# Autodesk Inventor assembly: Sestava1
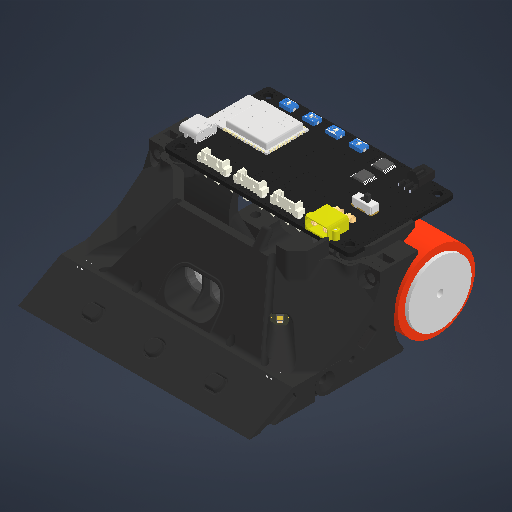
[picture p0: Inventor's stored thumbnail of the model, 512x512]
Saved by Autodesk Inventor 2025 (Build 290162000, 162)
## iProperties
Created: 2024-10-19
Part Number: Sestava1
Document SubType Name: Assembly
Designer: Simak
Author: Simak
## Documents named in this file (12)
- C:\_desktop\GitHub\Sumec-MiniSumo\-3D-\main_sumec_assembly.iam
- C:\_desktop\GitHub\Sumec-MiniSumo\-3D-\3D_printed\body-main.ipt
- C:\_desktop\GitHub\Sumec-MiniSumo\-3D-\3D_printed\body-front.ipt
- C:\_desktop\GitHub\Sumec-MiniSumo\-3D-\electronics\pololu-digital-distance-sensor-irs17a.ipt
- C:\_desktop\GitHub\Sumec-MiniSumo\-3D-\electronics\AssemBeneWake TF-LUNA.ipt
- C:\_desktop\GitHub\Sumec-MiniSumo\-3D-\electronics\PCBs\QRE MiniBoards\QRE MiniBoards\QRE_MiniBoards_Board.iam
- C:\_desktop\GitHub\Sumec-MiniSumo\-3D-\3D_printed\body-motor_comparment.ipt
- C:\_desktop\GitHub\Sumec-MiniSumo\-3D-\electronics\pololu_12v_650rpm-cb-enc-side-con.ipt
- C:\_desktop\GitHub\Sumec-MiniSumo\-3D-\machined\JSUMO_Wheel_33x25mm.ipt
- C:\_desktop\GitHub\Sumec-MiniSumo\-3D-\3D_printed\motor_C_clamp.ipt
- C:\_desktop\GitHub\Sumec-MiniSumo\-3D-\electronics\PCBs\main board\SUMEC_MK_IV.iam
- C:\_desktop\GitHub\Sumec-MiniSumo\-3D-\electronics\3s_lipo_small.ipt
## Components (12 placed, 11 different names)
1. body-main:1 — OPEN, Stejný směr:1, Vložit:1, Vložit:3, Proti sobě:6, Stejný směr:3, Proti sobě:7, Stejný směr:5, Vložit:6, Stejný směr:7, Vložit:7
2. body-front:1 — OPEN, Stejný směr:1, Vložit:1, Stejný směr:2, Proti sobě:2, Proti sobě:3, Proti sobě:4, Úhel:1, Tečnost:1, Vložit:2, Proti sobě:5
3. pololu-digital-distance-sensor-irs17a:1 — Stejný směr:2, Proti sobě:2, Proti sobě:3
4. AssemBeneWake TF-LUNA:1 — Proti sobě:4, Úhel:1, Tečnost:1
5. QRE_MiniBoards_Board:1 [sub-assembly] — Vložit:2, Proti sobě:5
6. pololu-digital-distance-sensor-irs17a:2 — Vložit:3, Proti sobě:6
7. body-motor_comparment:1 — Stejný směr:3, Proti sobě:7, Proti sobě:8, Proti sobě:9, Proti sobě:10, Proti sobě:11, Vložit:5, Stejný směr:6, Vložit:7
8. pololu_12v_650rpm-cb-enc-side-con:1 — Proti sobě:8, Proti sobě:9, Proti sobě:10, Vložit:4
9. JSUMO_Wheel_33x25mm:1 — Vložit:4, Stejný směr:5
10. motor_C_clamp:1 — Proti sobě:11, Vložit:5, Stejný směr:6
11. SUMEC_MK_IV:1 [sub-assembly] — Vložit:6, Stejný směr:7
12. 3s_lipo_small:1
## Relationships (26: Mate 11, Insert 7, Flush 6, Angle 1, Tangent 1)
- OPEN [Mate]: body-main:1 ↔ body-front:1
- Stejný směr:1 [Flush]: body-main:1 ↔ body-front:1
- Vložit:1 [Insert]: body-main:1 ↔ body-front:1
- Stejný směr:2 [Flush]: body-front:1 ↔ pololu-digital-distance-sensor-irs17a:1
- Proti sobě:2 [Mate]: body-front:1 ↔ pololu-digital-distance-sensor-irs17a:1
- Proti sobě:3 [Mate]: body-front:1 ↔ pololu-digital-distance-sensor-irs17a:1
- Proti sobě:4 [Mate]: body-front:1 ↔ AssemBeneWake TF-LUNA:1
- Úhel:1 [Angle] (0 deg): body-front:1 ↔ AssemBeneWake TF-LUNA:1
- Tečnost:1 [Tangent] (-0.1 mm): body-front:1 ↔ AssemBeneWake TF-LUNA:1
- Vložit:2 [Insert]: body-front:1 ↔ QRE_MiniBoards_Board:1
- Proti sobě:5 [Mate]: body-front:1 ↔ QRE_MiniBoards_Board:1
- Vložit:3 [Insert] (-0.5 mm): body-main:1 ↔ pololu-digital-distance-sensor-irs17a:2
- Proti sobě:6 [Mate]: body-main:1 ↔ pololu-digital-distance-sensor-irs17a:2
- Stejný směr:3 [Flush]: body-main:1 ↔ body-motor_comparment:1
- Proti sobě:7 [Mate] (0.25 mm): body-main:1 ↔ body-motor_comparment:1
- Proti sobě:8 [Mate]: body-motor_comparment:1 ↔ pololu_12v_650rpm-cb-enc-side-con:1
- Proti sobě:9 [Mate]: body-motor_comparment:1 ↔ pololu_12v_650rpm-cb-enc-side-con:1
- Proti sobě:10 [Mate]: body-motor_comparment:1 ↔ pololu_12v_650rpm-cb-enc-side-con:1
- Vložit:4 [Insert]: pololu_12v_650rpm-cb-enc-side-con:1 ↔ JSUMO_Wheel_33x25mm:1
- Stejný směr:5 [Flush]: body-main:1 ↔ JSUMO_Wheel_33x25mm:1
- Proti sobě:11 [Mate] (1 mm): body-motor_comparment:1 ↔ motor_C_clamp:1
- Vložit:5 [Insert]: body-motor_comparment:1 ↔ motor_C_clamp:1
- Stejný směr:6 [Flush]: body-motor_comparment:1 ↔ motor_C_clamp:1
- Vložit:6 [Insert]: body-main:1 ↔ SUMEC_MK_IV:1
- Stejný směr:7 [Flush]: body-main:1 ↔ SUMEC_MK_IV:1
- Vložit:7 [Insert]: body-main:1 ↔ body-motor_comparment:1
